# Autodesk Inventor assembly: LframeAssembly
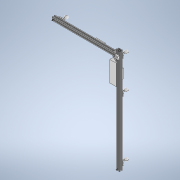
[picture p0: Inventor's stored thumbnail of the model, 180x180]
Saved by Autodesk Inventor 2022 (Build 260153000, 153)
## iProperties
Created: 2021-10-04
Part Number: LframeAssembly
Document SubType Name: Assembly
Designer: tecware
Author: tecware
## Documents named in this file (10)
- C:\Users\tecware\Documents\git\calibrationKit\L-frame\_LframeAssembly.iam
- C:\Users\tecware\Documents\git\calibrationKit\L-frame\components_L-frame\2020 Aluminum profile - 590mm.ipt
- C:\Users\tecware\Documents\git\calibrationKit\L-frame\components_L-frame\2020 Aluminum profile - 370mm.ipt
- C:\Users\tecware\Documents\git\calibrationKit\L-frame\components_L-frame\Corner Base Piece\corner.ipt
- C:\Users\tecware\Documents\git\calibrationKit\L-frame\components_L-frame\2020 Aluminum profile bracket.ipt
- C:\Users\tecware\Documents\git\calibrationKit\L-frame\components_L-frame\raisedMarkerWIthBase.ipt
- C:\Users\tecware\Documents\git\calibrationKit\L-frame\components_L-frame\M4 x 30mm Socket Head Screw.ipt
- C:\Users\tecware\Documents\git\calibrationKit\L-frame\components_L-frame\Enclosure\L Frame Enclosure.ipt
- C:\Users\tecware\Documents\git\calibrationKit\L-frame\components_L-frame\Enclosure\L Frame Enclosure Cover.ipt
- C:\Users\tecware\Documents\git\calibrationKit\L-frame\components_L-frame\Spirit Bubble Holder for L-frame\bubbleSpiritHolder - Lframe.ipt
## Components (20 placed, 9 different names)
1. 2020 Aluminum profile - 590mm:1 — Flush:1, Mate:2, Flush:3, Flush:4, Flush:14, Flush:15, Flush:16, Flush:19, Flush:20, Flush:21, Flush:22, Mate:14, Mate:16, Flush:25, Flush:26, Mate:18, Mate:19, Mate:20, Mate:24, Flush:27, Mate:29
2. 2020 Aluminum profile - 370mm:1 — Flush:1, Flush:17, Flush:18, Mate:13, Flush:24, Mate:14, Mate:17, Mate:21, Mate:22, Mate:28
3. corner:1 — Mate:2, Flush:3, Flush:4
4. raisedMarkerWIthBase:7 — Mate:5, Flush:6, Flush:7, Mate:23
5. raisedMarkerWIthBase:8 — Mate:5, Flush:6, Flush:7, Flush:17, Flush:18
6. raisedMarkerWIthBase:9 — markerToMarkerCenter, markerToMarkerSide, markerToMarkerTop, Mate:9
7. raisedMarkerWIthBase:10 — markerToMarkerCenter, markerToMarkerSide, markerToMarkerTop, Flush:14, Flush:15, Flush:16, Mate:23
8. raisedMarkerWIthBase:11 — Mate:10
9. raisedMarkerWIthBase:12 — Flush:19, Flush:20, Mate:9
10. raisedMarkerWIthBase:13
11. raisedMarkerWIthBase:14 — Flush:21, Flush:22, Mate:10
12. 2020 Aluminum profile bracket:3 — Flush:25, Flush:26, Mate:17, Mate:18
13. 2020 Aluminum profile bracket:4 — Mate:13, Flush:24, Mate:16
14. M4 x 30mm Socket Head Screw:1 — Mate:21, Mate:22
15. M4 x 30mm Socket Head Screw:2 — Mate:19, Mate:20
16. L Frame Enclosure:1 — Mate:24, Flush:27, Mate:25, Mate:26, Mate:27
17. L Frame Enclosure Cover:1 — Mate:25, Mate:26, Mate:27
18. bubbleSpiritHolder - Lframe:1 — Mate:28
19. bubbleSpiritHolder - Lframe:2 — Mate:29
20. bubbleSpiritHolder - Lframe:3
## Relationships (47: Flush 24, Mate 23)
- Flush:1: 2020 Aluminum profile - 590mm:1 ↔ 2020 Aluminum profile - 370mm:1
- Mate:2: 2020 Aluminum profile - 590mm:1 ↔ corner:1
- Flush:3 (20 mm): 2020 Aluminum profile - 590mm:1 ↔ corner:1
- Flush:4: 2020 Aluminum profile - 590mm:1 ↔ corner:1
- Mate:5: raisedMarkerWIthBase:7 ↔ raisedMarkerWIthBase:8
- Flush:6: raisedMarkerWIthBase:7 ↔ raisedMarkerWIthBase:8
- Flush:7: raisedMarkerWIthBase:7 ↔ raisedMarkerWIthBase:8
- markerToMarkerCenter [Mate]: raisedMarkerWIthBase:9 ↔ raisedMarkerWIthBase:10
- markerToMarkerSide [Flush]: raisedMarkerWIthBase:9 ↔ raisedMarkerWIthBase:10
- markerToMarkerTop [Flush]: raisedMarkerWIthBase:9 ↔ raisedMarkerWIthBase:10
- [Mate]: raisedMarkerWIthBase:11 ↔ raisedMarkerWIthBase:12
- [Flush]: raisedMarkerWIthBase:11 ↔ raisedMarkerWIthBase:12
- [Flush]: raisedMarkerWIthBase:11 ↔ raisedMarkerWIthBase:12
- [Mate]: raisedMarkerWIthBase:13 ↔ raisedMarkerWIthBase:14
- [Flush]: raisedMarkerWIthBase:13 ↔ raisedMarkerWIthBase:14
- [Flush]: raisedMarkerWIthBase:13 ↔ raisedMarkerWIthBase:14
- Flush:14 (15 mm): 2020 Aluminum profile - 590mm:1 ↔ raisedMarkerWIthBase:10
- Flush:15: 2020 Aluminum profile - 590mm:1 ↔ raisedMarkerWIthBase:10
- Flush:16 (-7 mm): 2020 Aluminum profile - 590mm:1 ↔ raisedMarkerWIthBase:10
- Flush:17: 2020 Aluminum profile - 370mm:1 ↔ raisedMarkerWIthBase:8
- Flush:18 (-7 mm): 2020 Aluminum profile - 370mm:1 ↔ raisedMarkerWIthBase:8
- Flush:19 (-7 mm): 2020 Aluminum profile - 590mm:1 ↔ raisedMarkerWIthBase:12
- Flush:20: 2020 Aluminum profile - 590mm:1 ↔ raisedMarkerWIthBase:12
- Flush:21: 2020 Aluminum profile - 590mm:1 ↔ raisedMarkerWIthBase:14
- Flush:22 (-7 mm): 2020 Aluminum profile - 590mm:1 ↔ raisedMarkerWIthBase:14
- Mate:9 (170 mm): raisedMarkerWIthBase:9 ↔ raisedMarkerWIthBase:12
- Mate:10 (336 mm): raisedMarkerWIthBase:11 ↔ raisedMarkerWIthBase:14
- Mate:13: 2020 Aluminum profile - 370mm:1 ↔ 2020 Aluminum profile bracket:4
- Flush:24: 2020 Aluminum profile - 370mm:1 ↔ 2020 Aluminum profile bracket:4
- Mate:14: 2020 Aluminum profile - 590mm:1 ↔ 2020 Aluminum profile - 370mm:1
- Mate:16: 2020 Aluminum profile - 590mm:1 ↔ 2020 Aluminum profile bracket:4
- Flush:25: 2020 Aluminum profile - 590mm:1 ↔ 2020 Aluminum profile bracket:3
- Flush:26: 2020 Aluminum profile - 590mm:1 ↔ 2020 Aluminum profile bracket:3
- Mate:17: 2020 Aluminum profile - 370mm:1 ↔ 2020 Aluminum profile bracket:3
- Mate:18: 2020 Aluminum profile - 590mm:1 ↔ 2020 Aluminum profile bracket:3
- Mate:19: 2020 Aluminum profile - 590mm:1 ↔ M4 x 30mm Socket Head Screw:2
- Mate:20: 2020 Aluminum profile - 590mm:1 ↔ M4 x 30mm Socket Head Screw:2
- Mate:21: 2020 Aluminum profile - 370mm:1 ↔ M4 x 30mm Socket Head Screw:1
- Mate:22: 2020 Aluminum profile - 370mm:1 ↔ M4 x 30mm Socket Head Screw:1
- Mate:23 (340 mm): raisedMarkerWIthBase:7 ↔ raisedMarkerWIthBase:10
- Mate:24: 2020 Aluminum profile - 590mm:1 ↔ L Frame Enclosure:1
- Flush:27: 2020 Aluminum profile - 590mm:1 ↔ L Frame Enclosure:1
- Mate:25 (0.1 mm): L Frame Enclosure:1 ↔ L Frame Enclosure Cover:1
- Mate:26 (7 mm): L Frame Enclosure:1 ↔ L Frame Enclosure Cover:1
- Mate:27 (0.2 mm): L Frame Enclosure:1 ↔ L Frame Enclosure Cover:1
- Mate:28: 2020 Aluminum profile - 370mm:1 ↔ bubbleSpiritHolder - Lframe:1
- Mate:29: 2020 Aluminum profile - 590mm:1 ↔ bubbleSpiritHolder - Lframe:2
## Named parameters: d12_d10 = 0 mm, d13_d11 = 0 mm, d14_d9 = 0 mm, d15_d12_d10 = 0 mm, d16_d13_d11 = 0 mm, d17_d14_d9 = 0 mm, d18_d12_d10 = 0 mm, d19_d13_d11 = 0 mm, d20_d14_d9 = 0 mm
